# Autodesk Inventor assembly: ExtendingArm_Adaptive
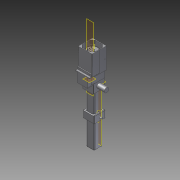
[picture p0: Inventor's stored thumbnail of the model, 180x180]
Saved by Autodesk Inventor 2012 (Build 160160000, 160)
## iProperties
Created: 2011-10-02
Part Number: ExtendingArm_Adaptive
Document SubType Name: Assembly
Designer: KuttaA
Mass: 266.79 g
Surface Area: 1474.69 cm^2
Volume: 266.518 cm^3
Density: 1.00102 g/cm^3
Author: KuttaA
## Documents named in this file (13)
- C:\Users\KuttaA\Dropbox\Hexapod Research\Leg Design\ExtendingArm_Adaptive.iam
- C:\Users\KuttaA\Dropbox\Hexapod Research\Leg Design\Screw.ipt
- C:\Users\KuttaA\Dropbox\Hexapod Research\Leg Design\LowerArm.ipt
- C:\Users\KuttaA\Dropbox\Hexapod Research\Leg Design\UpperRobotArm.ipt
- C:\Users\KuttaA\Dropbox\Hexapod Research\Leg Design\InternalKey.ipt
- C:\Users\KuttaA\Dropbox\Hexapod Research\Leg Design\ServoToScrewKey.ipt
- C:\Users\KuttaA\Dropbox\Hexapod Research\Leg Design\Other Parts\Motor.ipt
- C:\Users\KuttaA\Dropbox\Hexapod Research\Leg Design\Other Parts\MotorHousing.ipt
- C:\Users\KuttaA\Dropbox\Hexapod Research\Leg Design\Other Parts\Intermediary Gear Box\GearBox_ProperConstraints.iam
- C:\Users\KuttaA\Dropbox\Hexapod Research\Leg Design\Other Parts\Motor Housing\MotorHousingBottom.ipt
- C:\Users\KuttaA\Dropbox\Hexapod Research\Leg Design\Other Parts\ArmPivot.ipt
- C:\Users\KuttaA\Dropbox\Hexapod Research\Leg Design\Other Parts\Motor Housing\MotorHousingGearboxTop.ipt
- C:\Users\KuttaA\Dropbox\Hexapod Research\Leg Design\Other Parts\Motor Housing\MotorHousingTopMotorSupport.ipt
## Components (13 placed, 11 different names)
1. Screw:1 — Mate:1, Mate:2, Mate:3, Mate:8, Mate:9, Mate:10, Mate:21, Mate:30, Mate:31, Mate:32
2. LowerArm:1 — Mate:1, Mate:2, Mate:4, Mate:5
3. UpperRobotArm:1 — Mate:3, Mate:4, Mate:5, Mate:6, Mate:7, Flush:2, Mate:29, Flush:3
4. InternalKey:1 — Mate:6, Mate:7, Mate:29
5. MotorToScrewKey:1 — Mate:8, Mate:9, Mate:10
6. Motor:1 — Mate:21, Mate:34, Mate:36, Angle:37, Flush:5
7. ArmPivot:1 — Flush:2, Mate:37, Mate:38, Mate:39, Mate:40
8. GearBox_ProperConstraints:1 [sub-assembly] — Mate:30, Mate:31, Mate:32, Mate:34, Mate:36, Angle:37, Flush:6
9. ArmPivot:2 — Mate:37, Mate:38
10. MotorHousingBottom:1 — Flush:3, Flush:5, Flush:6, Flush:7, Flush:8, Flush:9, Flush:10
11. ArmPivot:3 — Mate:39, Mate:40
12. MotorHousingGearboxTop:1 — Flush:7, Flush:9, Flush:10
13. MotorHousingTopMotorSupport:1 — Flush:8
## Relationships (30: Mate 21, Flush 8, Angle 1)
- Mate:1: Screw:1 ↔ LowerArm:1
- Mate:2: Screw:1 ↔ LowerArm:1
- Mate:3 (0.3 mm): Screw:1 ↔ UpperRobotArm:1
- Mate:4 (0.3 mm): LowerArm:1 ↔ UpperRobotArm:1
- Mate:5 (0.3 mm): LowerArm:1 ↔ UpperRobotArm:1
- Mate:6 (0.3 mm): UpperRobotArm:1 ↔ InternalKey:1
- Mate:7 (0.3 mm): UpperRobotArm:1 ↔ InternalKey:1
- Mate:8 (0.3 mm): Screw:1 ↔ MotorToScrewKey:1
- Mate:9 (0.3 mm): Screw:1 ↔ MotorToScrewKey:1
- Mate:10 (0.3 mm): Screw:1 ↔ MotorToScrewKey:1
- Flush:2: UpperRobotArm:1 ↔ ArmPivot:1
- Mate:21 (13.5 mm): Screw:1 ↔ Motor:1
- Mate:29 (0.3 mm): UpperRobotArm:1 ↔ InternalKey:1
- Mate:30: Screw:1 ↔ GearBox_ProperConstraints:1
- Mate:31: Screw:1 ↔ GearBox_ProperConstraints:1
- Mate:32: Screw:1 ↔ GearBox_ProperConstraints:1
- Mate:34: Motor:1 ↔ GearBox_ProperConstraints:1
- Mate:36: Motor:1 ↔ GearBox_ProperConstraints:1
- Angle:37 (180 deg): Motor:1 ↔ GearBox_ProperConstraints:1
- Flush:3: UpperRobotArm:1 ↔ MotorHousingBottom:1
- Mate:37 (0.3 mm): ArmPivot:1 ↔ ArmPivot:2
- Mate:38: ArmPivot:1 ↔ ArmPivot:2
- Mate:39: ArmPivot:1 ↔ ArmPivot:3
- Mate:40 (0.3 mm): ArmPivot:1 ↔ ArmPivot:3
- Flush:5: Motor:1 ↔ MotorHousingBottom:1
- Flush:6: GearBox_ProperConstraints:1 ↔ MotorHousingBottom:1
- Flush:7: MotorHousingBottom:1 ↔ MotorHousingGearboxTop:1
- Flush:8: MotorHousingBottom:1 ↔ MotorHousingTopMotorSupport:1
- Flush:9: MotorHousingBottom:1 ↔ MotorHousingGearboxTop:1
- Flush:10: MotorHousingBottom:1 ↔ MotorHousingGearboxTop:1
